# Autodesk Inventor assembly: RB4
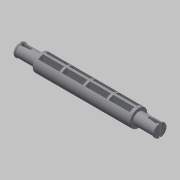
[picture p0: Inventor's stored thumbnail of the model, 180x180]
Saved by Autodesk Inventor 2019.3 (Build 233278000, 278)
## iProperties
Created: 2019-02-05
Part Number: RB4
Document SubType Name: Assembly
Designer: Varga Daniel
Author: Varga Daniel
## Documents named in this file (5)
- C:\!_Dani\!_cloud\OneDrive\!_munka\Revolution\RevvyDemoKit\Structural parts\Beams\Round Beams\RB1+\RB4.iam
- C:\!_Dani\!_cloud\OneDrive\!_munka\Revolution\RevvyDemoKit\Structural parts\Beams\Round Beams\Round_beam_body.ipt
- C:\!_Dani\!_cloud\OneDrive\!_munka\Revolution\RevvyDemoKit\Structural parts\Connetor Pins\Connector_pin_collar.ipt
- C:\!_Dani\!_cloud\OneDrive\!_munka\Revolution\RevvyDemoKit\Structural parts\Connetor Pins\Connector_pin_stick.ipt
- C:\!_Dani\!_cloud\OneDrive\!_munka\Revolution\RevvyDemoKit\Structural parts\Beams\Round Beams\RB1+.iam
## Components (8 placed, 3 different names)
1. Connector_pin_collar:1 — Mate:3, Mate:4, Mate:7, Mate:8
2. Connector_pin_stick:1 — Mate:3, Mate:4, Angle:1, Angle:4
3. Connector_pin_collar:2 — Mate:1, Mate:2, Mate:5, Mate:6, Mate:7, Mate:8
4. Connector_pin_stick:2 — Mate:1, Mate:2, Angle:1, Angle:2, Angle:3, Angle:4
5. Round_beam_body:2 — Mate:5, Mate:6, Angle:3
6. Round_beam_body:3
7. Round_beam_body:4
8. Round_beam_body:5
## Component patterns: (4 elements, first: Round_beam_body:2)
## Relationships (12: Mate 8, Angle 4)
- Mate:1: Connector_pin_collar:2 ↔ Connector_pin_stick:2
- Mate:2: Connector_pin_collar:2 ↔ Connector_pin_stick:2
- Mate:3: Connector_pin_collar:1 ↔ Connector_pin_stick:1
- Mate:4: Connector_pin_collar:1 ↔ Connector_pin_stick:1
- Angle:1 (0 deg): Connector_pin_stick:1 ↔ Connector_pin_stick:2
- Angle:2 (0 deg): Connector_pin_stick:2
- Mate:5: Connector_pin_collar:2 ↔ Round_beam_body:2
- Mate:6: Connector_pin_collar:2 ↔ Round_beam_body:2
- Angle:3 (0 deg): Connector_pin_stick:2 ↔ Round_beam_body:2
- Mate:7 (40 mm): Connector_pin_collar:1 ↔ Connector_pin_collar:2
- Mate:8: Connector_pin_collar:1 ↔ Connector_pin_collar:2
- Angle:4 (0 deg): Connector_pin_stick:1 ↔ Connector_pin_stick:2
